# Autodesk Inventor assembly: Assembly3
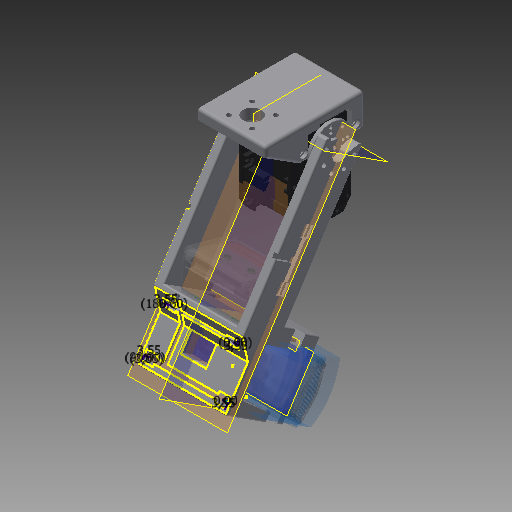
[picture p0: Inventor's stored thumbnail of the model, 512x512]
Saved by Autodesk Inventor 2018 (Build 220112000, 112)
## iProperties
Created: 2018-05-16
Part Number: Assembly3
Document SubType Name: Assembly
Designer: bitbots
Author: bitbots
## Documents named in this file (7)
- C:\Users\jaspe\gits\bitbots_hardware\wolfgang\assembly\head\head.iam
- head.iam
- C:\Users\jaspe\gits\bitbots_hardware\wolfgang\assembly\head\Logitech_C910_(interior).ipt
- C:\Users\jaspe\gitss\bitbots_hardware\wolfgang\assembly\head\camera_holder.ipt
- C:\Users\jaspe\gits\bitbots_hardware\wolfgang\assembly\motors\MX64\Mx64_with_bearing.iam
- C:\Users\jaspe\gits\bitbots_hardware\wolfgang\assembly\head\hals.ipt
- C:\Users\jaspe\gits\bitbots_hardware\wolfgang\assembly\head\head_calibration.ipt
## Components (5 placed, 5 different names)
1. Logitech_C910_(interior):1 — Flush:1, Flush:2, Flush:3
2. camera_holder:1 — Flush:1, Flush:2, Flush:3, Flush:12, Mate:15
3. Mx64_with_bearing:1 [sub-assembly] — Mate:7, Flush:11, Mate:13, Mate:14
4. hals:1 — Mate:7, Flush:11
5. head_calibration:1 — Flush:12, Mate:13, Mate:14, Mate:15
## Relationships (9: Flush 5, Mate 4)
- Flush:1: Logitech_C910_(interior):1 ↔ camera_holder:1
- Flush:2 (1 mm): Logitech_C910_(interior):1 ↔ camera_holder:1
- Flush:3 (1 mm): Logitech_C910_(interior):1 ↔ camera_holder:1
- Mate:7 (0.5 mm): Mx64_with_bearing:1 ↔ hals:1
- Flush:11 (-17 mm): Mx64_with_bearing:1 ↔ hals:1
- Flush:12: camera_holder:1 ↔ head_calibration:1
- Mate:13: Mx64_with_bearing:1 ↔ head_calibration:1
- Mate:14: Mx64_with_bearing:1 ↔ head_calibration:1
- Mate:15: camera_holder:1 ↔ head_calibration:1
